# Autodesk Inventor assembly: dog_2
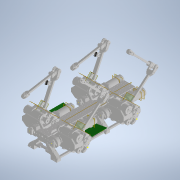
[picture p0: Inventor's stored thumbnail of the model, 180x180]
Saved by Autodesk Inventor 2020 (Build 240168000, 168)
## iProperties
Created: 2019-05-16
Part Number: dog_2
Document SubType Name: Assembly
Designer: psrob
Author: psrob
## Documents named in this file (16)
- E:\projects-2\project dog gen2\hardware\dog_2.iam
- E:\projects-2\project dog gen2\hardware\leg_ass_1.iam
- E:\projects-2\project dog gen2\hardware\carbon_fiber_200.ipt
- E:\projects-2\project dog gen2\hardware\leg_ass_1_MIR.iam
- E:\projects-2\project dog gen2\hardware\body_bone_1.ipt
- E:\projects-2\project dog gen2\hardware\body_bone_2.ipt
- E:\projects-2\project dog gen2\hardware\body_bone_3.ipt
- E:\projects-2\project dog gen2\hardware\body_bone_4.ipt
- E:\projects-2\project dog gen2\hardware\body_bone_5.ipt
- E:\projects-2\project dog gen2\hardware\body_carbon_fiber_holder_1.ipt
- E:\projects-2\project dog gen2\hardware\pcb_holder_1.ipt
- E:\projects-2\project dog gen2\hardware\pcb_holder_2.ipt
- E:\projects-2\project dog gen2\hardware\ele_3d_2\dog_driver_4.brd.iam
- E:\projects-2\project dog gen2\hardware\motor_holder_1.ipt
- E:\projects-2\project dog gen2\hardware\pcb_holder_4.ipt
- E:\projects-2\project dog gen2\hardware\pcb_holder_4_MIR.ipt
## Components (27 placed, 15 different names)
1. leg_ass_1:1 [sub-assembly] — Flush:2, Flush:3, Flush:4, Mate:4, Flush:8, Flush:9, Insert:6, Flush:14, Insert:8
2. leg_ass_1:2 [sub-assembly] — Flush:2, Flush:3, Flush:4, Mate:1, Mate:2, Flush:5, Mate:3, Flush:6, Flush:7, Flush:10, Flush:12, Insert:1, Insert:4, Insert:10, Insert:11, Flush:27, Flush:32
3. carbon_fiber_200:1 — Mate:1, Mate:2, Flush:5, Flush:15, Flush:16
4. leg_ass_1_MIR:1 [sub-assembly] — Mate:3, Flush:6, Flush:7, Insert:2, Insert:3, Flush:13, Insert:9, Insert:12, Flush:31
5. leg_ass_1_MIR:2 [sub-assembly] — Mate:4, Flush:8, Flush:9, Flush:11, Insert:5, Insert:7
6. body_bone_1:1 — Flush:10, Insert:3, Insert:4, Insert:17, Insert:18, Insert:23, Insert:24
7. body_bone_2:1 — Flush:11, Insert:5, Insert:6, Insert:19, Insert:20, Insert:21, Insert:22
8. body_bone_3:1 — Flush:12, Insert:1, Insert:2
9. body_bone_4:1 — Flush:13, Insert:9, Insert:10, Insert:13, Insert:14
10. body_bone_5:1 — Flush:14, Insert:7, Insert:8, Mate:11
11. carbon_fiber_200:2 — Flush:15, Flush:16
12. body_bone_1:2 — Insert:11, Insert:12, Insert:15, Insert:16, Flush:28, Angle:1, Angle:2
13. body_carbon_fiber_holder_1:1 — Flush:27, Insert:13, Insert:14, Mate:12, Flush:29, Mate:13, Flush:30, Mate:14, Mate:15
14. body_carbon_fiber_holder_1:2 — Insert:15, Insert:16
15. pcb_holder_1:1 — Flush:28, Mate:16, Flush:33, Insert:25, Insert:26, Flush:35, Mate:17
16. pcb_holder_2:1 — Mate:11
17. carbon_fiber_200:3 — Mate:13, Flush:30, Mate:14
18. carbon_fiber_200:4 — Mate:12, Flush:29, Mate:15
19. dog_driver_4.brd:1 [sub-assembly] — Flush:32, Angle:2, Symmetry:1, Symmetry:2
20. dog_driver_4.brd:2 [sub-assembly] — Flush:31, Angle:1, Symmetry:1, Symmetry:2, Tangent:1, Mate:16
21. motor_holder_1:1 — Insert:17, Insert:18
22. motor_holder_1:2 — Insert:19, Insert:20
23. motor_holder_1:3 — Insert:23, Insert:24, Tangent:1
24. motor_holder_1:4 — Insert:21, Insert:22
25. pcb_holder_4:1 — Flush:33
26. pcb_holder_4_MIR:1 — Insert:25, Insert:26, Flush:34
27. pcb_holder_4_MIR:2 — Flush:34, Flush:35, Mate:17
## Relationships (66: Insert 26, Flush 24, Mate 11, Angle 2, Symmetry 2, Tangent 1)
- Flush:2: leg_ass_1:1 ↔ leg_ass_1:2
- Flush:3 (180 mm): leg_ass_1:1 ↔ leg_ass_1:2
- Flush:4: leg_ass_1:1 ↔ leg_ass_1:2
- Mate:1: leg_ass_1:2 ↔ carbon_fiber_200:1
- Mate:2: leg_ass_1:2 ↔ carbon_fiber_200:1
- Flush:5 (10 mm): leg_ass_1:2 ↔ carbon_fiber_200:1
- Mate:3: leg_ass_1:2 ↔ leg_ass_1_MIR:1
- Flush:6: leg_ass_1:2 ↔ leg_ass_1_MIR:1
- Flush:7: leg_ass_1:2 ↔ leg_ass_1_MIR:1
- Mate:4: leg_ass_1:1 ↔ leg_ass_1_MIR:2
- Flush:8: leg_ass_1:1 ↔ leg_ass_1_MIR:2
- Flush:9: leg_ass_1:1 ↔ leg_ass_1_MIR:2
- Flush:10: leg_ass_1:2 ↔ body_bone_1:1
- Flush:11: leg_ass_1_MIR:2 ↔ body_bone_2:1
- Flush:12: leg_ass_1:2 ↔ body_bone_3:1
- Insert:1: leg_ass_1:2 ↔ body_bone_3:1
- Insert:2: leg_ass_1_MIR:1 ↔ body_bone_3:1
- Insert:3: leg_ass_1_MIR:1 ↔ body_bone_1:1
- Insert:4: leg_ass_1:2 ↔ body_bone_1:1
- Insert:5: leg_ass_1_MIR:2 ↔ body_bone_2:1
- Insert:6: leg_ass_1:1 ↔ body_bone_2:1
- Flush:13: leg_ass_1_MIR:1 ↔ body_bone_4:1
- Flush:14: leg_ass_1:1 ↔ body_bone_5:1
- Insert:7: leg_ass_1_MIR:2 ↔ body_bone_5:1
- Insert:8: leg_ass_1:1 ↔ body_bone_5:1
- Insert:9: leg_ass_1_MIR:1 ↔ body_bone_4:1
- Insert:10: leg_ass_1:2 ↔ body_bone_4:1
- Flush:15: carbon_fiber_200:1 ↔ carbon_fiber_200:2
- Flush:16: carbon_fiber_200:1 ↔ carbon_fiber_200:2
- Insert:11: leg_ass_1:2 ↔ body_bone_1:2
- Insert:12: leg_ass_1_MIR:1 ↔ body_bone_1:2
- Flush:27: leg_ass_1:2 ↔ body_carbon_fiber_holder_1:1
- Insert:13: body_bone_4:1 ↔ body_carbon_fiber_holder_1:1
- Insert:14: body_bone_4:1 ↔ body_carbon_fiber_holder_1:1
- Insert:15: body_bone_1:2 ↔ body_carbon_fiber_holder_1:2
- Insert:16: body_bone_1:2 ↔ body_carbon_fiber_holder_1:2
- Flush:28: body_bone_1:2 ↔ pcb_holder_1:1
- Mate:11: body_bone_5:1 ↔ pcb_holder_2:1
- Mate:12: body_carbon_fiber_holder_1:1 ↔ carbon_fiber_200:4
- Flush:29: body_carbon_fiber_holder_1:1 ↔ carbon_fiber_200:4
- Mate:13: body_carbon_fiber_holder_1:1 ↔ carbon_fiber_200:3
- Flush:30: body_carbon_fiber_holder_1:1 ↔ carbon_fiber_200:3
- Mate:14: body_carbon_fiber_holder_1:1 ↔ carbon_fiber_200:3
- Mate:15: body_carbon_fiber_holder_1:1 ↔ carbon_fiber_200:4
- Flush:31 (15 mm): leg_ass_1_MIR:1 ↔ dog_driver_4.brd:2
- Angle:1 (170 deg): body_bone_1:2 ↔ dog_driver_4.brd:2
- Flush:32 (15 mm): leg_ass_1:2 ↔ dog_driver_4.brd:1
- Angle:2 (190 deg): body_bone_1:2 ↔ dog_driver_4.brd:1
- Symmetry:1: dog_driver_4.brd:1 ↔ dog_driver_4.brd:2
- Symmetry:2: dog_driver_4.brd:1 ↔ dog_driver_4.brd:2
- Insert:17: body_bone_1:1 ↔ motor_holder_1:1
- Insert:18: body_bone_1:1 ↔ motor_holder_1:1
- Insert:19: body_bone_2:1 ↔ motor_holder_1:2
- Insert:20: body_bone_2:1 ↔ motor_holder_1:2
- Insert:21: body_bone_2:1 ↔ motor_holder_1:4
- Insert:22: body_bone_2:1 ↔ motor_holder_1:4
- Insert:23: body_bone_1:1 ↔ motor_holder_1:3
- Insert:24: body_bone_1:1 ↔ motor_holder_1:3
- Tangent:1 (1 mm): dog_driver_4.brd:2 ↔ motor_holder_1:3
- Mate:16 (5 mm): pcb_holder_1:1 ↔ dog_driver_4.brd:2
- Flush:33: pcb_holder_1:1 ↔ pcb_holder_4:1
- Insert:25: pcb_holder_1:1 ↔ pcb_holder_4_MIR:1
- Insert:26: pcb_holder_1:1 ↔ pcb_holder_4_MIR:1
- Flush:34: pcb_holder_4_MIR:1 ↔ pcb_holder_4_MIR:2
- Flush:35: pcb_holder_1:1 ↔ pcb_holder_4_MIR:2
- Mate:17: pcb_holder_1:1 ↔ pcb_holder_4_MIR:2
